# Autodesk Inventor assembly: Plunger Assembly
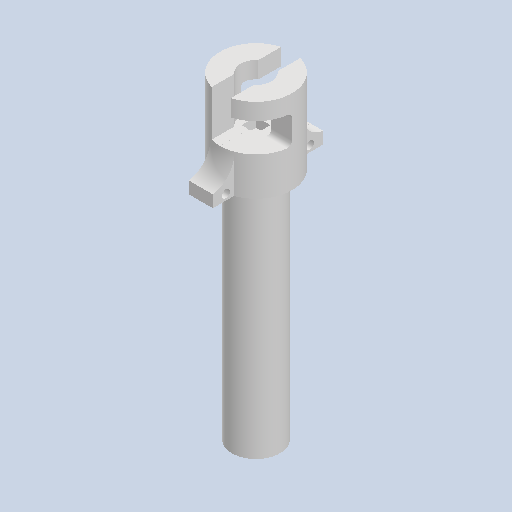
[picture p0: Inventor's stored thumbnail of the model, 512x512]
Saved by Autodesk Inventor 2022 (Build 260153000, 153)
## iProperties
Created: 2021-12-01
Part Number: Plunger Assembly
Document SubType Name: Assembly
Designer: efred
Author: efred
## Documents named in this file (3)
- C:\Users\efred\OneDrive - Imperial College London\ROBOICP\Final Assembly\Plunger Assembly.iam
- C:\Users\efred\OneDrive - Imperial College London\ROBOICP\Final Assembly\Syringe Plunger.ipt
- C:\Users\efred\OneDrive - Imperial College London\ROBOICP\Final Assembly\Syringe Lock.ipt
## Components (3 placed, 2 different names)
1. Syringe Plunger:1 — Mate:1, Mate:2, Mate:3
2. Syringe Lock:1 — Mate:1, Mate:2, Mate:3
3. Syringe Lock:2
## Component patterns: (2 elements, first: Syringe Lock:1)
## Relationships (3: Mate 3)
- Mate:1: Syringe Plunger:1 ↔ Syringe Lock:1
- Mate:2 (0.1 mm): Syringe Plunger:1 ↔ Syringe Lock:1
- Mate:3: Syringe Plunger:1 ↔ Syringe Lock:1
